# Autodesk Inventor assembly: DD_KVD_004
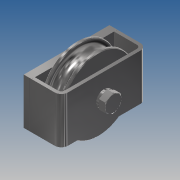
[picture p0: Inventor's stored thumbnail of the model, 180x180]
Saved by Autodesk Inventor 2017.3 (Build 213256000, 256)
## iProperties
Created: 2023-12-15
Part Number: DD_KVD_004
Document SubType Name: Assembly
Designer: Darena
Author: Darena
## iProperties of the stored document groove_ball_bearing_-_6201-2rs1_0_02.ipt
Created: 2012-07-27
Part Number: groove_ball_bearing_-_6201-2rs1_0_02
Checked By: TraceParts S.A.
Material: Všeobecné
Catalog Web Link: www.traceparts.com
Document SubType Name: Modeling
Designer: TraceParts
Mass: 0.121395 g
Surface Area: 8.20794 cm^2
Volume: 0.121395 cm^3
Density: 1 g/cm^3
Appearance: Výchozí
Company: TraceParts S.A.
Author: TraceParts
Sending System: Autodesk Inventor 2018
## iProperties of the stored document groove_ball_bearing_-_6201-2rs1_0_03.ipt
Created: 2012-07-27
Part Number: groove_ball_bearing_-_6201-2rs1_0_03
Checked By: TraceParts S.A.
Material: Všeobecné
Catalog Web Link: www.traceparts.com
Document SubType Name: Modeling
Designer: TraceParts
Mass: 2.38515 g
Surface Area: 14.3109 cm^2
Volume: 2.38515 cm^3
Density: 1 g/cm^3
Appearance: Výchozí
Company: TraceParts S.A.
Author: TraceParts
Sending System: Autodesk Inventor 2018
## iProperties of the stored document groove_ball_bearing_-_6201-2rs1_0.iam
Company: TraceParts S.A.
Created: 2012-07-27
Part Number: 6201-2RS1
Checked By: TraceParts S.A.
Catalog Web Link: www.traceparts.com
Description: Single row deep groove ball bearing with seals - for shaft Ø12
Vendor: SKF
Document SubType Name: Assembly
Designer: TraceParts
Mass: 5.54086 g
Surface Area: 64.9817 cm^2
Volume: 5.54086 cm^3
Density: 1 g/cm^3
Title: Single row deep groove ball bearing with seals - for shaft Ø12
Author: TraceParts
Sending System: Autodesk Inventor 2018
DESIGN: Single row deep groove ball bearing with seals - for shaft Ø12
REFERENCE: 6201-2RS1
MASS: 0,04 kg
SUPPLIER: SKF
STANDARD: ISO 15-1981, BS 6267
## iProperties of the stored document groove_ball_bearing_-_6201-2rs1_0_05.ipt
Created: 2012-07-27
Part Number: groove_ball_bearing_-_6201-2rs1_0_05
Checked By: TraceParts S.A.
Material: Všeobecné
Catalog Web Link: www.traceparts.com
Document SubType Name: Modeling
Designer: TraceParts
Mass: 1.9626 g
Surface Area: 23.3167 cm^2
Volume: 1.9626 cm^3
Density: 1 g/cm^3
Appearance: Výchozí
Company: TraceParts S.A.
Author: TraceParts
Sending System: Autodesk Inventor 2018
## iProperties of the stored document groove_ball_bearing_-_6201-2rs1_0_01.ipt
Created: 2012-07-27
Part Number: groove_ball_bearing_-_6201-2rs1_0_01
Checked By: TraceParts S.A.
Material: Všeobecné
Catalog Web Link: www.traceparts.com
Document SubType Name: Modeling
Designer: TraceParts
Mass: 0.121395 g
Surface Area: 8.20794 cm^2
Volume: 0.121395 cm^3
Density: 1 g/cm^3
Appearance: Výchozí
Company: TraceParts S.A.
Author: TraceParts
Sending System: Autodesk Inventor 2018
## iProperties of the stored document groove_ball_bearing_-_6201-2rs1_0_04.ipt
Created: 2012-07-27
Part Number: groove_ball_bearing_-_6201-2rs1_0_04
Checked By: TraceParts S.A.
Material: Všeobecné
Catalog Web Link: www.traceparts.com
Document SubType Name: Modeling
Designer: TraceParts
Mass: 0.950319 g
Surface Area: 10.9382 cm^2
Volume: 0.950319 cm^3
Density: 1 g/cm^3
Appearance: Výchozí
Company: TraceParts S.A.
Author: TraceParts
Sending System: Autodesk Inventor 2018
## Documents named in this file (20)
- **D:\2_Darena\1_Soukrome\02_Inventor soukromé\Dílna RAKO3\Záhora\Pivovar KONTEJNER\S výklopným dnem\DD_KVD_001\DD_KVD_004.iam*LocalDocs*xJwqdjizdMntded0sW3tos1i4Ng*groove_ball_bearing_-_6201-2rs1_0_02.ipt
- **D:\2_Darena\1_Soukrome\02_Inventor soukromé\Dílna RAKO3\Záhora\Pivovar KONTEJNER\S výklopným dnem\DD_KVD_001\DD_KVD_004.iam*LocalDocs*xFn4maui5HmgnusciTpdfn1fk4b*groove_ball_bearing_-_6201-2rs1_0_03.ipt
- **D:\2_Darena\1_Soukrome\02_Inventor soukromé\Dílna RAKO3\Záhora\Pivovar KONTEJNER\S výklopným dnem\DD_KVD_001\DD_KVD_004.iam*LocalDocs*x2g3g1bqhIid5u5odNkie1l3xJe*groove_ball_bearing_-_6201-2rs1_0.iam
- **D:\2_Darena\1_Soukrome\02_Inventor soukromé\Dílna RAKO3\Záhora\Pivovar KONTEJNER\S výklopným dnem\DD_KVD_001\DD_KVD_004.iam*LocalDocs*xQxiv21g2WgcduqwoT0vevzxjFd*groove_ball_bearing_-_6201-2rs1_0_05.ipt
- **D:\2_Darena\1_Soukrome\02_Inventor soukromé\Dílna RAKO3\Záhora\Pivovar KONTEJNER\S výklopným dnem\DD_KVD_001\DD_KVD_004.iam*LocalDocs*xXpemb3bj1nsxeqkwTetrc2ygDd*groove_ball_bearing_-_6201-2rs1_0_04.ipt
- **D:\2_Darena\1_Soukrome\02_Inventor soukromé\Dílna RAKO3\Záhora\Pivovar KONTEJNER\S výklopným dnem\DD_KVD_001\DD_KVD_004.iam*LocalDocs*xMxunzm30Zxtnel4fGqh4ydc43d*groove_ball_bearing_-_6201-2rs1_0_01.ipt
- D:\2_Darena\1_Soukrome\02_Inventor soukromé\Dílna RAKO3\Záhora\Pivovar KONTEJNER\S výklopným dnem\DD_KVD_001\DD_KVD_004.iam
- D:\2_Darena\1_Soukrome\02_Inventor soukromé\Dílna RAKO3\Záhora\Pivovar KONTEJNER\S výklopným dnem\DD_KVD_001\DD_KVD_004_02.ipt
- D:\2_Darena\1_Soukrome\02_Inventor soukromé\Dílna RAKO3\Záhora\Pivovar KONTEJNER\S výklopným dnem\DD_KVD_001\DD_KVD_004_03.ipt
- D:\2_Darena\1_Soukrome\02_Inventor soukromé\Dílna RAKO3\Záhora\Pivovar KONTEJNER\S výklopným dnem\DD_KVD_001\DD_KVD_004_04.iam
- D:\2_Darena\1_Soukrome\02_Inventor soukromé\Dílna RAKO3\Záhora\Pivovar KONTEJNER\S výklopným dnem\DD_KVD_001\DD_KVD_004_05.ipt
- D:\2_Darena\1_Soukrome\02_Inventor soukromé\Dílna RAKO3\Záhora\Pivovar KONTEJNER\S výklopným dnem\DD_KVD_001\DD_KVD_004_06.ipt
- D:\2_Darena\1_Soukrome\02_Inventor soukromé\Dílna RAKO3\Záhora\Pivovar KONTEJNER\S výklopným dnem\DD_KVD_001\CSN 02 1740 - 8.ipt
- D:\2_Darena\1_Soukrome\02_Inventor soukromé\Dílna RAKO3\Záhora\Pivovar KONTEJNER\S výklopným dnem\DD_KVD_001\CSN 02 1201 - M8 x 1,25 x 30.ipt
- D:\2_Darena\1_Soukrome\02_Inventor soukromé\Dílna RAKO3\Záhora\Pivovar KONTEJNER\S výklopným dnem\DD_KVD_001\6201-2RS\groove_ball_bearing_-_6201-2rs1_0.iam
- D:\2_Darena\1_Soukrome\02_Inventor soukromé\Dílna RAKO3\Záhora\Pivovar KONTEJNER\S výklopným dnem\DD_KVD_001\6201-2RS\groove_ball_bearing_-_6201-2rs1_0_01.ipt
- D:\2_Darena\1_Soukrome\02_Inventor soukromé\Dílna RAKO3\Záhora\Pivovar KONTEJNER\S výklopným dnem\DD_KVD_001\6201-2RS\groove_ball_bearing_-_6201-2rs1_0_02.ipt
- D:\2_Darena\1_Soukrome\02_Inventor soukromé\Dílna RAKO3\Záhora\Pivovar KONTEJNER\S výklopným dnem\DD_KVD_001\6201-2RS\groove_ball_bearing_-_6201-2rs1_0_03.ipt
- D:\2_Darena\1_Soukrome\02_Inventor soukromé\Dílna RAKO3\Záhora\Pivovar KONTEJNER\S výklopným dnem\DD_KVD_001\6201-2RS\groove_ball_bearing_-_6201-2rs1_0_04.ipt
- D:\2_Darena\1_Soukrome\02_Inventor soukromé\Dílna RAKO3\Záhora\Pivovar KONTEJNER\S výklopným dnem\DD_KVD_001\6201-2RS\groove_ball_bearing_-_6201-2rs1_0_05.ipt
## Components (8 placed, 8 different names)
1. DD_KVD_004_02:1 — Proti sobě:1, Stejný směr:1, Vložit:2, Proti sobě:4
2. DD_KVD_004_03:1 — Proti sobě:1, Proti sobě:2, Proti sobě:3, Stejný směr:1, Vložit:1, Proti sobě:5
3. DD_KVD_004_04:1 [sub-assembly] — Proti sobě:2, Proti sobě:3, Vložit:3, Úhel:1
4. DD_KVD_004_05:1 — Vložit:1
5. DD_KVD_004_06:1 — Vložit:2
6. groove_ball_bearing_-_6201-2rs1_0:1 [sub-assembly] — Proti sobě:4, Proti sobě:5
7. CSN 02 1740 - 8:1 — Vložit:3, Vložit:4
8. CSN 02 1201 - M8 x 1,25 x 30:1 — Vložit:4, Úhel:1
## Relationships (11: Mate 5, Insert 4, Flush 1, Angle 1)
- Proti sobě:1 [Mate]: DD_KVD_004_02:1 ↔ DD_KVD_004_03:1
- Proti sobě:2 [Mate]: DD_KVD_004_03:1 ↔ DD_KVD_004_04:1
- Proti sobě:3 [Mate]: DD_KVD_004_03:1 ↔ DD_KVD_004_04:1
- Stejný směr:1 [Flush]: DD_KVD_004_02:1 ↔ DD_KVD_004_03:1
- Vložit:1 [Insert]: DD_KVD_004_03:1 ↔ DD_KVD_004_05:1
- Vložit:2 [Insert]: DD_KVD_004_02:1 ↔ DD_KVD_004_06:1
- Proti sobě:4 [Mate]: DD_KVD_004_02:1 ↔ groove_ball_bearing_-_6201-2rs1_0:1
- Proti sobě:5 [Mate]: DD_KVD_004_03:1 ↔ groove_ball_bearing_-_6201-2rs1_0:1
- Vložit:3 [Insert]: DD_KVD_004_04:1 ↔ CSN 02 1740 - 8:1
- Vložit:4 [Insert]: CSN 02 1740 - 8:1 ↔ CSN 02 1201 - M8 x 1,25 x 30:1
- Úhel:1 [Angle] (0 deg): DD_KVD_004_04:1 ↔ CSN 02 1201 - M8 x 1,25 x 30:1
